# Autodesk Inventor assembly: LIA0007-NETWORKING SHELF
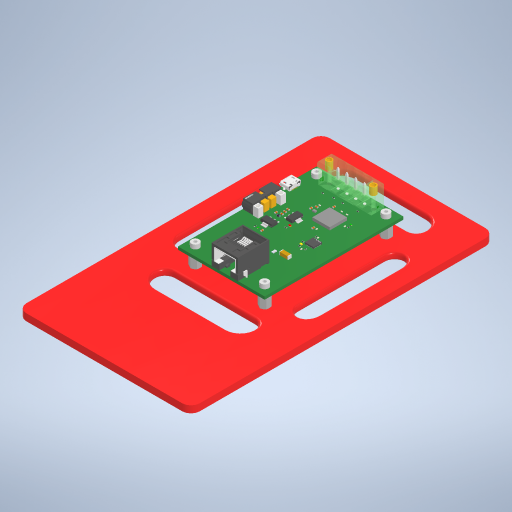
[picture p0: Inventor's stored thumbnail of the model, 512x512]
Saved by Autodesk Inventor 2023 (Build 270158000, 158)
## iProperties
Created: 2023-05-24
Part Number: LIA0007-NETWORKING SHELF
Document SubType Name: Assembly
Designer: Louis
Author: Louis
## Documents named in this file (6)
- D:\Louis\Documents\Inventor\Interferometry\LIA0007-NETWORKING SHELF.iam
- D:\Louis\Documents\Inventor\Interferometry\LI0018-NETWORKING SHELF.ipt
- D:\Louis\Documents\Inventor\Interferometry\ACCU HHTPS-M2.5-5-8-S-Z.ipt
- D:\Louis\Documents\Inventor\Interferometry\AltiumPIC32_PCB.iam
- D:\Louis\Documents\Inventor\Interferometry\M2.5 X 6.ipt
- D:\Louis\Documents\Inventor\Interferometry\M2.5 WASHER.ipt
## Components (18 placed, 5 different names)
1. LI0018-NETWORKING SHELF:1 — Mate:1, Mate:2, Flush:1, Insert:1, Insert:2, Insert:3, Insert:4, Insert:13, Insert:14, Insert:15, Insert:16
2. ACCU HHTPS-M2.5-5-8-S-Z:1 — Insert:3, Insert:6
3. ACCU HHTPS-M2.5-5-8-S-Z:2 — Insert:4, Insert:8
4. ACCU HHTPS-M2.5-5-8-S-Z:3 — Insert:2, Insert:5
5. ACCU HHTPS-M2.5-5-8-S-Z:4 — Insert:1, Insert:7
6. AltiumPIC32_PCB:1 [sub-assembly] — Insert:5, Insert:6, Insert:7, Insert:8, Insert:9, Insert:10, Insert:11, Insert:12
7. M2.5 X 6:1 — Insert:9
8. M2.5 X 6:2 — Insert:10
9. M2.5 X 6:3 — Insert:17
10. M2.5 X 6:4 — Insert:11
11. M2.5 X 6:5 — Insert:20
12. M2.5 X 6:6 — Insert:12
13. M2.5 X 6:7 — Insert:19
14. M2.5 X 6:8 — Insert:18
15. M2.5 WASHER:1 — Insert:13, Insert:17
16. M2.5 WASHER:2 — Insert:16, Insert:20
17. M2.5 WASHER:3 — Insert:15, Insert:19
18. M2.5 WASHER:4 — Insert:14, Insert:18
## Relationships (23: Insert 20, Mate 2, Flush 1)
- Mate:1: LI0018-NETWORKING SHELF:1
- Mate:2: LI0018-NETWORKING SHELF:1
- Flush:1: LI0018-NETWORKING SHELF:1
- Insert:1: LI0018-NETWORKING SHELF:1 ↔ ACCU HHTPS-M2.5-5-8-S-Z:4
- Insert:2: LI0018-NETWORKING SHELF:1 ↔ ACCU HHTPS-M2.5-5-8-S-Z:3
- Insert:3: LI0018-NETWORKING SHELF:1 ↔ ACCU HHTPS-M2.5-5-8-S-Z:1
- Insert:4: LI0018-NETWORKING SHELF:1 ↔ ACCU HHTPS-M2.5-5-8-S-Z:2
- Insert:5: ACCU HHTPS-M2.5-5-8-S-Z:3 ↔ AltiumPIC32_PCB:1
- Insert:6: ACCU HHTPS-M2.5-5-8-S-Z:1 ↔ AltiumPIC32_PCB:1
- Insert:7: ACCU HHTPS-M2.5-5-8-S-Z:4 ↔ AltiumPIC32_PCB:1
- Insert:8: ACCU HHTPS-M2.5-5-8-S-Z:2 ↔ AltiumPIC32_PCB:1
- Insert:9: AltiumPIC32_PCB:1 ↔ M2.5 X 6:1
- Insert:10: AltiumPIC32_PCB:1 ↔ M2.5 X 6:2
- Insert:11: AltiumPIC32_PCB:1 ↔ M2.5 X 6:4
- Insert:12: AltiumPIC32_PCB:1 ↔ M2.5 X 6:6
- Insert:13: LI0018-NETWORKING SHELF:1 ↔ M2.5 WASHER:1
- Insert:14: LI0018-NETWORKING SHELF:1 ↔ M2.5 WASHER:4
- Insert:15: LI0018-NETWORKING SHELF:1 ↔ M2.5 WASHER:3
- Insert:16: LI0018-NETWORKING SHELF:1 ↔ M2.5 WASHER:2
- Insert:17: M2.5 X 6:3 ↔ M2.5 WASHER:1
- Insert:18: M2.5 X 6:8 ↔ M2.5 WASHER:4
- Insert:19: M2.5 X 6:7 ↔ M2.5 WASHER:3
- Insert:20: M2.5 X 6:5 ↔ M2.5 WASHER:2
